# Autodesk Inventor assembly: Overall_assembly_new
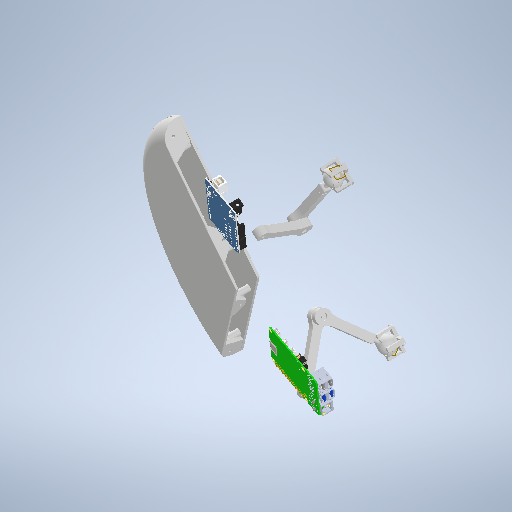
[picture p0: Inventor's stored thumbnail of the model, 512x512]
Saved by Autodesk Inventor 2025.1 (Build 291241000, 241)
## iProperties
Created: 2024-11-10
Part Number: Overall_assembly_new
Document SubType Name: Assembly
Designer: xingj
Author: xingj
## Documents named in this file (13)
- C:\Users\zombulli\OneDrive - Carl Zeiss AG\Desktop\DHBW\Semester 5\mte380\CAD\Stewart Platform\Overall_assembly_new.iam
- C:\Users\zombulli\OneDrive - Carl Zeiss AG\Desktop\DHBW\Semester 5\mte380\CAD\Stewart Platform\Custom parts\Baseplate.ipt
- C:\Users\zombulli\OneDrive - Carl Zeiss AG\Desktop\DHBW\Semester 5\mte380\CAD\Stewart Platform\Custom parts\alternativeJoint - Kopie.ipt
- C:\Users\zombulli\OneDrive - Carl Zeiss AG\Desktop\DHBW\Semester 5\mte380\CAD\Stewart Platform\Custom parts\alternativeJoint2 - Kopie.ipt
- C:\Users\zombulli\OneDrive - Carl Zeiss AG\Desktop\DHBW\Semester 5\mte380\CAD\Stewart Platform\Standard parts\dowel.ipt
- C:\Users\zombulli\OneDrive - Carl Zeiss AG\Desktop\DHBW\Semester 5\mte380\CAD\Stewart Platform\Custom parts\balljoint_male.ipt
- C:\Users\zombulli\OneDrive - Carl Zeiss AG\Desktop\DHBW\Semester 5\mte380\CAD\Stewart Platform\Custom parts\female_1,3.ipt
- C:\Users\zombulli\OneDrive - Carl Zeiss AG\Desktop\DHBW\Semester 5\mte380\CAD\Stewart Platform\Custom parts\clip_1,3.ipt
- C:\Users\zombulli\OneDrive - Carl Zeiss AG\Desktop\DHBW\Semester 5\mte380\CAD\Stewart Platform\Custom parts\platform balancing plate.ipt
- C:\Users\zombulli\OneDrive - Carl Zeiss AG\Desktop\DHBW\Semester 5\mte380\CAD\Stewart Platform\arduino uno\arduino uno\arduino uno.ipt
- C:\Users\zombulli\OneDrive - Carl Zeiss AG\Desktop\DHBW\Semester 5\mte380\CAD\Stewart Platform\Raspberry Pi\Raspberry Pi 4 Model B\Raspberry Pi 4 Model B\Raspberry Pi 4 Model B.ipt
- C:\Users\zombulli\OneDrive - Carl Zeiss AG\Desktop\DHBW\Semester 5\mte380\CAD\Stewart Platform\stepper_new.ipt
- C:\Users\zombulli\OneDrive - Carl Zeiss AG\Desktop\DHBW\Semester 5\mte380\CAD\Stewart Platform\Custom parts\cover.ipt
## Components (25 placed, 12 different names)
1. Baseplate:1 — Passend:1, Passend:2, Passend:3, Passend:4, Passend:103, Passend:105, Passend:107, Fluchtend:11, Fluchtend:12, Passend:114
2. Baseplate:2 — Passend:1, Passend:2, Passend:5, Passend:101
3. Baseplate:3 — Passend:3, Passend:4, Passend:5, Passend:100
4. alternativeJoint - Kopie:1 — Passend:63, Passend:69
5. alternativeJoint2 - Kopie:1 — Passend:63, Passend:68, Fluchtend:1, Passend:82, Passend:83, Passend:84
6. dowel:2 — Passend:68, Passend:69, Fluchtend:1
7. dowel:3 — Passend:71, Passend:72, Passend:73, Fluchtend:2
8. alternativeJoint - Kopie:2 — Passend:70, Passend:73
9. alternativeJoint2 - Kopie:2 — Passend:70, Passend:71, Passend:72, Fluchtend:2, Passend:85, Passend:86, Passend:87
10. alternativeJoint - Kopie:3 — Passend:108, Passend:109, Passend:110, Passend:111
11. balljoint_male:1 — Passend:82, Passend:83, Passend:84, Kugelförmig:3
12. balljoint_male:2 — Passend:112, Passend:113, Fluchtend:10
13. balljoint_male:3 — Passend:85, Passend:86, Passend:87, Kugelförmig:1
14. female_1,3:1 — Kugelförmig:1, Fluchtend:4, Passend:88, Fluchtend:5, Passend:95, Passend:99
15. clip_1,3:3 — Fluchtend:6, Passend:92, Fluchtend:7
16. female_1,3:2 — Kugelförmig:3, Fluchtend:8, Passend:93, Fluchtend:9, Passend:96, Passend:98
17. female_1,3:3 — Fluchtend:6, Passend:92, Fluchtend:7, Passend:94, Passend:97
18. clip_1,3:4 — Fluchtend:8, Passend:93, Fluchtend:9
19. clip_1,3:5 — Fluchtend:4, Passend:88, Fluchtend:5
20. platform balancing plate:1 — Passend:94, Passend:95, Passend:96, Passend:97, Passend:98, Passend:99
21. arduino uno:1 — Passend:100
22. Raspberry Pi 4 Model B:1 — Passend:101
23. stepper_new:1 — Passend:103, Passend:105, Passend:107, Passend:108, Passend:109
24. alternativeJoint2 - Kopie:3 — Passend:110, Passend:111, Passend:112, Passend:113, Fluchtend:10
25. cover:1 — Fluchtend:11, Fluchtend:12, Passend:114
## Relationships (52: Mate 39, Flush 11, BallJoint 2)
- Passend:1 [Mate]: Baseplate:1 ↔ Baseplate:2
- Passend:2 [Mate]: Baseplate:1 ↔ Baseplate:2
- Passend:3 [Mate]: Baseplate:1 ↔ Baseplate:3
- Passend:4 [Mate]: Baseplate:1 ↔ Baseplate:3
- Passend:5 [Mate]: Baseplate:2 ↔ Baseplate:3
- Passend:63 [Mate]: alternativeJoint - Kopie:1 ↔ alternativeJoint2 - Kopie:1
- Passend:68 [Mate]: alternativeJoint2 - Kopie:1 ↔ dowel:2
- Passend:69 [Mate]: alternativeJoint - Kopie:1 ↔ dowel:2
- Fluchtend:1 [Flush]: alternativeJoint2 - Kopie:1 ↔ dowel:2
- Passend:70 [Mate]: alternativeJoint - Kopie:2 ↔ alternativeJoint2 - Kopie:2
- Passend:71 [Mate]: dowel:3 ↔ alternativeJoint2 - Kopie:2
- Passend:72 [Mate]: dowel:3 ↔ alternativeJoint2 - Kopie:2
- Passend:73 [Mate]: dowel:3 ↔ alternativeJoint - Kopie:2
- Fluchtend:2 [Flush]: dowel:3 ↔ alternativeJoint2 - Kopie:2
- Passend:82 [Mate]: alternativeJoint2 - Kopie:1 ↔ balljoint_male:1
- Passend:83 [Mate]: alternativeJoint2 - Kopie:1 ↔ balljoint_male:1
- Passend:84 [Mate]: alternativeJoint2 - Kopie:1 ↔ balljoint_male:1
- Passend:85 [Mate]: alternativeJoint2 - Kopie:2 ↔ balljoint_male:3
- Passend:86 [Mate]: alternativeJoint2 - Kopie:2 ↔ balljoint_male:3
- Passend:87 [Mate]: alternativeJoint2 - Kopie:2 ↔ balljoint_male:3
- Kugelförmig:1 [BallJoint]: balljoint_male:3 ↔ female_1,3:1
- Fluchtend:4 [Flush]: female_1,3:1 ↔ clip_1,3:5
- Passend:88 [Mate]: female_1,3:1 ↔ clip_1,3:5
- Fluchtend:5 [Flush]: female_1,3:1 ↔ clip_1,3:5
- Fluchtend:6 [Flush]: clip_1,3:3 ↔ female_1,3:3
- Passend:92 [Mate]: clip_1,3:3 ↔ female_1,3:3
- Fluchtend:7 [Flush]: clip_1,3:3 ↔ female_1,3:3
- Kugelförmig:3 [BallJoint]: balljoint_male:1 ↔ female_1,3:2
- Fluchtend:8 [Flush]: female_1,3:2 ↔ clip_1,3:4
- Passend:93 [Mate]: female_1,3:2 ↔ clip_1,3:4
- Fluchtend:9 [Flush]: female_1,3:2 ↔ clip_1,3:4
- Passend:94 [Mate]: female_1,3:3 ↔ platform balancing plate:1
- Passend:95 [Mate]: female_1,3:1 ↔ platform balancing plate:1
- Passend:96 [Mate]: female_1,3:2 ↔ platform balancing plate:1
- Passend:97 [Mate]: female_1,3:3 ↔ platform balancing plate:1
- Passend:98 [Mate]: female_1,3:2 ↔ platform balancing plate:1
- Passend:99 [Mate]: female_1,3:1 ↔ platform balancing plate:1
- Passend:100 [Mate]: Baseplate:3 ↔ arduino uno:1
- Passend:101 [Mate]: Baseplate:2 ↔ Raspberry Pi 4 Model B:1
- Passend:103 [Mate]: Baseplate:1 ↔ stepper_new:1
- Passend:105 [Mate]: Baseplate:1 ↔ stepper_new:1
- Passend:107 [Mate]: Baseplate:1 ↔ stepper_new:1
- Passend:108 [Mate] (0.5 mm): alternativeJoint - Kopie:3 ↔ stepper_new:1
- Passend:109 [Mate]: alternativeJoint - Kopie:3 ↔ stepper_new:1
- Passend:110 [Mate]: alternativeJoint - Kopie:3 ↔ alternativeJoint2 - Kopie:3
- Passend:111 [Mate]: alternativeJoint - Kopie:3 ↔ alternativeJoint2 - Kopie:3
- Passend:112 [Mate]: balljoint_male:2 ↔ alternativeJoint2 - Kopie:3
- Passend:113 [Mate]: balljoint_male:2 ↔ alternativeJoint2 - Kopie:3
- Fluchtend:10 [Flush]: balljoint_male:2 ↔ alternativeJoint2 - Kopie:3
- Fluchtend:11 [Flush]: Baseplate:1 ↔ cover:1
- Fluchtend:12 [Flush]: Baseplate:1 ↔ cover:1
- Passend:114 [Mate]: Baseplate:1 ↔ cover:1
